# Autodesk Inventor assembly: rat_enclosure
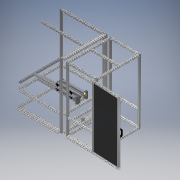
[picture p0: Inventor's stored thumbnail of the model, 180x180]
Saved by Autodesk Inventor 2019 (Build 230136000, 136)
## iProperties
Created: 2018-07-19
Part Number: rat_enclosure
Document SubType Name: Assembly
Designer: Brian
Author: Brian
## Documents named in this file (29)
- C:\Users\bgereke\Desktop\designs\rat_enclosure.iam
- C:\Users\bgereke\Desktop\designs\24in_1010.ipt
- C:\Users\bgereke\Desktop\designs\24in_1020.ipt
- C:\Users\bgereke\Desktop\designs\38in_1010.ipt
- C:\Users\bgereke\Desktop\designs\38in_1020.ipt
- C:\Users\bgereke\Desktop\designs\35in_1010.ipt
- C:\Users\bgereke\Desktop\designs\24in_half_1010.ipt
- C:\Users\bgereke\Desktop\designs\4in_1010.ipt
- C:\Users\bgereke\Desktop\designs\16in_1010.ipt
- C:\Users\bgereke\Desktop\designs\rat_enclosure_top_panel.ipt
- C:\Users\bgereke\Desktop\designs\rat_enclosure_side_panels.ipt
- C:\Users\bgereke\Desktop\designs\rat_enclosure_door_panel.ipt
- C:\Users\bgereke\Desktop\designs\16in_1020.ipt
- C:\Users\bgereke\Desktop\designs\16in_half_1010.ipt
- C:\Users\bgereke\Desktop\designs\arm_enclosure_back_panel.ipt
- C:\Users\bgereke\Desktop\designs\arm_enclosure_top_panel.ipt
- C:\Users\bgereke\Desktop\designs\arm_enclosure_side_panel.ipt
- C:\Users\bgereke\Desktop\designs\arm_enclosure_door_panel.ipt
- C:\Users\bgereke\Desktop\designs\2062\2062.ipt
- C:\Users\bgereke\Desktop\designs\rat_enclosure_slide_panel.ipt
- C:\Users\bgereke\Documents\BSE poster 2019\Gimbal_bot.iam
- C:\Users\bgereke\Desktop\designs\Nord\BRAIN-assembly-complete-model-08-13-18.iam
- C:\Users\bgereke\Desktop\designs\head port\head_port_1.ipt
- C:\Users\bgereke\Desktop\designs\8020_27511\AIS2019\2751-1.iam
- C:\Users\bgereke\Desktop\designs\4in_1020.ipt
- C:\Users\bgereke\Desktop\designs\3310T592_STRUT CHANNEL.ipt
- C:\Users\bgereke\Desktop\designs\confiner_back_panel.ipt
- C:\Users\bgereke\Desktop\designs\confiner_floor.ipt
- C:\Users\bgereke\Desktop\designs\confiner_sliding_panel.ipt
## Components (77 placed, 28 different names)
1. 24in_1010:1 — Flush:3, Mate:5, Mate:6, Flush:12, Flush:14, Mate:18, Flush:45
2. 24in_1010:3 — Flush:3, Mate:5, Mate:6, Flush:13, Flush:25
3. 24in_1020:1 — Flush:25, Flush:34, Mate:30, Flush:104, Flush:166, Mate:114, Mate:150
4. 24in_1010:4 — Mate:17, Mate:20, Flush:36, Flush:37, Mate:31, Flush:42, Flush:130
5. 24in_1010:6 — Flush:22, Flush:28, Mate:26, Mate:27, Flush:29, Flush:131, Mate:134
6. 24in_1020:2 — Mate:25, Flush:30, Flush:35, Flush:57, Mate:82, Mate:102, Mate:132
7. 38in_1010:3 — Flush:12, Flush:13, Flush:14, Flush:22, Mate:20, Flush:27, Mate:24, Mate:27, Flush:129, Mate:88, Mate:156, Flush:196
8. 24in_1010:7 — Mate:17, Mate:18, Flush:20, Flush:27, Mate:24, Flush:43, Mate:87, Mate:182, Flush:234
9. 24in_1010:8 — Flush:20, Flush:33, Mate:29, Flush:73, Flush:272
10. 38in_1020:1 — Flush:28, Mate:25, Mate:26, Flush:29, Flush:30, Flush:33, Flush:34, Mate:29, Flush:35, Mate:30, Flush:74, Flush:100
11. 38in_1020:2 — Flush:36, Flush:37, Mate:31, Flush:40, Flush:41, Mate:33, Mate:34, Flush:46, Mate:35, Flush:54
12. 24in_1010:9 — Flush:40, Flush:41, Flush:42, Mate:33, Flush:55, Flush:56, Flush:177, Mate:133
13. 24in_1010:10 — Flush:43, Mate:34, Flush:54
14. 24in_1020:3 — Flush:45, Flush:46, Mate:35
15. 24in_half_1010:2 — Flush:132, Mate:90, Mate:145
16. 24in_half_1010:1
17. 35in_1010:1 — Mate:91, Mate:144, Flush:183
18. 35in_1010:2
19. 38in_1010:4 — Flush:55, Flush:56, Flush:57, Mate:51, Mate:81, Mate:83, Mate:84, Mate:86
20. 24in_1020:4 — Flush:73, Flush:74, Mate:51, Mate:85, Mate:150, Mate:151, Flush:188, Flush:277, Flush:282, Mate:226
21. 38in_1010:6 — Flush:100, Flush:108, Mate:69, Flush:109, Flush:120, Flush:121, Flush:136, Mate:98, Flush:140, Flush:144
22. 24in_1010:11 — Mate:98, Flush:140, Flush:144, Mate:102, Flush:145, Flush:147, Flush:163
23. 24in_1010:12 — Flush:104, Flush:157, Flush:158, Flush:166, Mate:114
24. 16in_1010:2 — Flush:108, Mate:69, Flush:109
25. 38in_1010:8 — Mate:72, Flush:117, Mate:75, Flush:124, Mate:78, Mate:96, Flush:151, Flush:153, Flush:154, Flush:155, Mate:117, Mate:118, Mate:119
26. 24in_1010:13 — Mate:72, Flush:150, Flush:151, Mate:104, Flush:161, Mate:116, Flush:174, Mate:135
27. 24in_1010:14 — Flush:117, Flush:155, Flush:156, Mate:118, Mate:120, Mate:121
28. 16in_1010:4 — Flush:120, Flush:121, Mate:75, Flush:135, Mate:105, Flush:153, Mate:137
29. 16in_1010:5 — Flush:123, Flush:126, Mate:79, Mate:80, Mate:107, Flush:160, Flush:164
30. 16in_1010:6 — Flush:123, Flush:124, Mate:78
31. 24in_1010:15 — Flush:126, Mate:79, Flush:127, Flush:186
32. 24in_1010:16 — Flush:127, Mate:80, Mate:148, Flush:185
33. rat_enclosure_top_panel:1 — Mate:81, Mate:82, Mate:83
34. rat_enclosure_top_panel:2 — Mate:84, Mate:85, Mate:86, Mate:149, Flush:187
35. rat_enclosure_side_panels:1 — Flush:129, Flush:130, Mate:87, Mate:89
36. rat_enclosure_side_panels:2 — Flush:131, Mate:88, Mate:89
37. rat_enclosure_door_panel:1 — Flush:132, Mate:90, Mate:91
38. arm_enclosure_back_panel:1 — Flush:135, Mate:96, Flush:136, Mate:105, Flush:154
39. 16in_1020:1 — Flush:156, Mate:106, Flush:159, Mate:110, Mate:112, Angle:4
40. 38in_1020:4 — Flush:150, Mate:104, Mate:106, Flush:159, Mate:107, Flush:160, Flush:162, Mate:113, Flush:169
41. 38in_1010:9 — Flush:145, Flush:147, Flush:157, Flush:158, Flush:164, Flush:165, Mate:108
42. 16in_1010:7 — Flush:161, Flush:162, Flush:163, Flush:165, Mate:108, Flush:178, Mate:136
43. 35in_1010:3 — Flush:167, Flush:168, Mate:111, Flush:170
44. 16in_half_1010:1 — Mate:110, Flush:167, Flush:168, Mate:111, Mate:112, Mate:113, Angle:4, Flush:171, Mate:123, Mate:125
45. 16in_half_1010:2 — Flush:169, Flush:170, Flush:171, Flush:172, Mate:115, Flush:173, Mate:143
46. 35in_1010:4 — Flush:172, Mate:115, Flush:173, Mate:124, Mate:142, Flush:182
47. arm_enclosure_top_panel:1 — Mate:116, Flush:174, Mate:117
48. arm_enclosure_side_panel:1 — Mate:119, Mate:120, Mate:121
49. arm_enclosure_door_panel:1 — Mate:123, Mate:124, Mate:125
50. 4in_1010:5
51. 4in_1010:6
52. 24in_1010:17 — Flush:177, Mate:132, Mate:133, Mate:134
53. 16in_1010:8 — Flush:178, Mate:135, Mate:136, Mate:137
54. 2062:1 — Mate:142, Flush:182, Mate:143
55. 2062:2 — Mate:144, Flush:183, Mate:145
56. rat_enclosure_slide_panel:1
57. Gimbal_bot:1 [sub-assembly] — Mate:148, Flush:185, Flush:186
58. BRAIN-assembly-complete-model-08-13-18:1 [sub-assembly] — Mate:149, Flush:187
59. 24in_1010:19 — Mate:151, Flush:188, Flush:252, Flush:272, Mate:242, Mate:243, Flush:298
60. 24in_1010:23 — Mate:156, Flush:196, Mate:227, Flush:283
61. head_port_1:1 — Flush:208, Flush:252, Mate:212, Flush:254, Mate:221, Flush:276, Mate:230, Flush:287
62. head_port_1:2 — Flush:208, Flush:253, Mate:212, Flush:254, Flush:255, Mate:225, Flush:289
63. 24in_1010:24 — Mate:182, Flush:234, Flush:253, Flush:255, Mate:234, Flush:290, Flush:297
64. 2751-1:1 [sub-assembly] — Flush:269, Mate:235, Mate:236, Flush:292
65. 2751-1:2 [sub-assembly] — Flush:269, Mate:237, Flush:293
66. 4in_1010:9 — Mate:221, Flush:276, Flush:277, Flush:281, Mate:228, Mate:239
67. 4in_1010:10 — Mate:233, Mate:234, Flush:290, Flush:292, Flush:293
68. 4in_1020:1 — Flush:281, Flush:282, Mate:225, Mate:226, Flush:284
69. 24in_1010:25 — Mate:227, Flush:283, Flush:284, Mate:235, Mate:236, Mate:237, Flush:291
70. 3310T592_STRUT CHANNEL:1 — Mate:228, Mate:230, Flush:287, Flush:288, Flush:294, Mate:238, Mate:244, Mate:245, Mate:247
71. 3310T592_STRUT CHANNEL:2 — Flush:288, Flush:289, Mate:233, Flush:291, Flush:295, Mate:240, Flush:296
72. confiner_back_panel:1 — Flush:294, Mate:238, Mate:239
73. confiner_back_panel:2 — Flush:295, Mate:240, Flush:296, Flush:299
74. confiner_floor:1 — Flush:297, Mate:242
75. 4in_1020:2 — Mate:243, Mate:244, Flush:298, Mate:246
76. confiner_sliding_panel:1 — Mate:245, Mate:246, Mate:247, Mate:248, Flush:300
77. confiner_sliding_panel:2 — Mate:248, Flush:299, Flush:300
## Relationships (229: Flush 120, Mate 106, Angle 3)
- Flush:3: 24in_1010:1 ↔ 24in_1010:3
- Mate:5: 24in_1010:1 ↔ 24in_1010:3
- Mate:6: 24in_1010:1 ↔ 24in_1010:3
- [Flush]: 24in_1010:4 ↔ 24in_1010:6
- [Mate]: 24in_1010:4 ↔ 24in_1010:6
- [Mate]: 24in_1010:4 ↔ 24in_1010:6
- Flush:12: 24in_1010:1 ↔ 38in_1010:3
- Flush:13: 24in_1010:3 ↔ 38in_1010:3
- Flush:14: 24in_1010:1 ↔ 38in_1010:3
- Mate:17: 24in_1010:4 ↔ 24in_1010:7
- Mate:18: 24in_1010:1 ↔ 24in_1010:7
- Flush:20: 24in_1010:7 ↔ 24in_1010:8
- Flush:22: 24in_1010:6 ↔ 38in_1010:3
- Mate:20: 24in_1010:4 ↔ 38in_1010:3
- Flush:25: 24in_1010:3 ↔ 24in_1020:1
- Flush:27: 38in_1010:3 ↔ 24in_1010:7
- Mate:24: 38in_1010:3 ↔ 24in_1010:7
- Flush:28: 24in_1010:6 ↔ 38in_1020:1
- Mate:25: 24in_1020:2 ↔ 38in_1020:1
- Mate:26: 24in_1010:6 ↔ 38in_1020:1
- Mate:27: 24in_1010:6 ↔ 38in_1010:3
- Flush:29: 24in_1010:6 ↔ 38in_1020:1
- Flush:30: 24in_1020:2 ↔ 38in_1020:1
- Flush:33: 24in_1010:8 ↔ 38in_1020:1
- Flush:34: 24in_1020:1 ↔ 38in_1020:1
- Mate:29: 24in_1010:8 ↔ 38in_1020:1
- Flush:35: 24in_1020:2 ↔ 38in_1020:1
- Mate:30: 24in_1020:1 ↔ 38in_1020:1
- Flush:36: 24in_1010:4 ↔ 38in_1020:2
- Flush:37: 24in_1010:4 ↔ 38in_1020:2
- Mate:31: 24in_1010:4 ↔ 38in_1020:2
- Flush:40: 38in_1020:2 ↔ 24in_1010:9
- Flush:41: 38in_1020:2 ↔ 24in_1010:9
- Flush:42: 24in_1010:4 ↔ 24in_1010:9
- Mate:33: 38in_1020:2 ↔ 24in_1010:9
- Flush:43: 24in_1010:7 ↔ 24in_1010:10
- Mate:34: 38in_1020:2 ↔ 24in_1010:10
- Flush:45: 24in_1010:1 ↔ 24in_1020:3
- Flush:46: 38in_1020:2 ↔ 24in_1020:3
- Mate:35: 38in_1020:2 ↔ 24in_1020:3
- [Flush]: 24in_1010:9 ↔ 24in_half_1010:2
- [Flush]: 24in_half_1010:2 ↔ 24in_half_1010:1
- [Flush]: 24in_half_1010:2 ↔ 24in_half_1010:1
- [Mate]: 24in_1020:3 ↔ 24in_half_1010:1
- [Mate] (1.778 mm): 38in_1020:2 ↔ 24in_half_1010:1
- [Angle] (0 deg): 24in_1020:3 ↔ 24in_half_1010:1
- [Angle] (0 deg): 24in_1020:3 ↔ 24in_half_1010:1
- [Flush]: 24in_half_1010:2 ↔ 35in_1010:1
- [Flush]: 24in_half_1010:2 ↔ 35in_1010:1
- [Mate]: 24in_half_1010:2 ↔ 35in_1010:1
- [Mate]: 24in_half_1010:1 ↔ 35in_1010:2
- [Flush]: 24in_half_1010:2 ↔ 35in_1010:2
- [Flush]: 24in_half_1010:2 ↔ 35in_1010:2
- Flush:54: 38in_1020:2 ↔ 24in_1010:10
- Flush:55: 24in_1010:9 ↔ 38in_1010:4
- Flush:56: 24in_1010:9 ↔ 38in_1010:4
- Flush:57: 24in_1020:2 ↔ 38in_1010:4
- Flush:73: 24in_1010:8 ↔ 24in_1020:4
- Flush:74: 38in_1020:1 ↔ 24in_1020:4
- Mate:51: 38in_1010:4 ↔ 24in_1020:4
- Flush:100: 38in_1020:1 ↔ 38in_1010:6
- Flush:104: 24in_1020:1 ↔ 24in_1010:12
- Flush:108: 38in_1010:6 ↔ 16in_1010:2
- Mate:69: 38in_1010:6 ↔ 16in_1010:2
- Flush:109: 38in_1010:6 ↔ 16in_1010:2
- Mate:72: 38in_1010:8 ↔ 24in_1010:13
- Flush:117: 38in_1010:8 ↔ 24in_1010:14
- Flush:120: 38in_1010:6 ↔ 16in_1010:4
- Flush:121: 38in_1010:6 ↔ 16in_1010:4
- Mate:75: 38in_1010:8 ↔ 16in_1010:4
- Flush:123: 16in_1010:5 ↔ 16in_1010:6
- Flush:124: 38in_1010:8 ↔ 16in_1010:6
- Mate:78: 38in_1010:8 ↔ 16in_1010:6
- Flush:126: 16in_1010:5 ↔ 24in_1010:15
- Mate:79: 16in_1010:5 ↔ 24in_1010:15
- Flush:127: 24in_1010:15 ↔ 24in_1010:16
- Mate:80: 16in_1010:5 ↔ 24in_1010:16
- Mate:81: 38in_1010:4 ↔ rat_enclosure_top_panel:1
- Mate:82: 24in_1020:2 ↔ rat_enclosure_top_panel:1
- Mate:83: 38in_1010:4 ↔ rat_enclosure_top_panel:1
- Mate:84: 38in_1010:4 ↔ rat_enclosure_top_panel:2
- Mate:85: 24in_1020:4 ↔ rat_enclosure_top_panel:2
- Mate:86: 38in_1010:4 ↔ rat_enclosure_top_panel:2
- Flush:129: 38in_1010:3 ↔ rat_enclosure_side_panels:1
- Flush:130: 24in_1010:4 ↔ rat_enclosure_side_panels:1
- Mate:87: 24in_1010:7 ↔ rat_enclosure_side_panels:1
- Flush:131: 24in_1010:6 ↔ rat_enclosure_side_panels:2
- Mate:88: 38in_1010:3 ↔ rat_enclosure_side_panels:2
- Mate:89: rat_enclosure_side_panels:1 ↔ rat_enclosure_side_panels:2
- Flush:132: 24in_half_1010:2 ↔ rat_enclosure_door_panel:1
- Mate:90: 24in_half_1010:2 ↔ rat_enclosure_door_panel:1
- Mate:91: 35in_1010:1 ↔ rat_enclosure_door_panel:1
- Flush:135: 16in_1010:4 ↔ arm_enclosure_back_panel:1
- Mate:96: 38in_1010:8 ↔ arm_enclosure_back_panel:1
- Flush:136: 38in_1010:6 ↔ arm_enclosure_back_panel:1
- Mate:98: 38in_1010:6 ↔ 24in_1010:11
- Flush:140: 38in_1010:6 ↔ 24in_1010:11
- Flush:144: 38in_1010:6 ↔ 24in_1010:11
- Mate:102: 24in_1020:2 ↔ 24in_1010:11
- Flush:145: 24in_1010:11 ↔ 38in_1010:9
- Flush:147: 24in_1010:11 ↔ 38in_1010:9
- Flush:150: 24in_1010:13 ↔ 38in_1020:4
- Flush:151: 38in_1010:8 ↔ 24in_1010:13
- Mate:104: 24in_1010:13 ↔ 38in_1020:4
- Mate:105: 16in_1010:4 ↔ arm_enclosure_back_panel:1
- Flush:153: 38in_1010:8 ↔ 16in_1010:4
- Flush:154: 38in_1010:8 ↔ arm_enclosure_back_panel:1
- Flush:155: 38in_1010:8 ↔ 24in_1010:14
- Flush:156: 24in_1010:14 ↔ 16in_1020:1
- Flush:157: 24in_1010:12 ↔ 38in_1010:9
- Flush:158: 24in_1010:12 ↔ 38in_1010:9
- Mate:106: 16in_1020:1 ↔ 38in_1020:4
- Flush:159: 16in_1020:1 ↔ 38in_1020:4
- Mate:107: 16in_1010:5 ↔ 38in_1020:4
- Flush:160: 16in_1010:5 ↔ 38in_1020:4
- Flush:161: 24in_1010:13 ↔ 16in_1010:7
- Flush:162: 38in_1020:4 ↔ 16in_1010:7
- Flush:163: 24in_1010:11 ↔ 16in_1010:7
- Flush:164: 16in_1010:5 ↔ 38in_1010:9
- Flush:165: 38in_1010:9 ↔ 16in_1010:7
- Mate:108: 38in_1010:9 ↔ 16in_1010:7
- Flush:166: 24in_1020:1 ↔ 24in_1010:12
- Mate:110: 16in_1020:1 ↔ 16in_half_1010:1
- Flush:167: 35in_1010:3 ↔ 16in_half_1010:1
- Flush:168: 35in_1010:3 ↔ 16in_half_1010:1
- Mate:111: 35in_1010:3 ↔ 16in_half_1010:1
- Mate:112: 16in_1020:1 ↔ 16in_half_1010:1
- Mate:113 (2.54 mm): 38in_1020:4 ↔ 16in_half_1010:1
- Angle:4 (0 deg): 16in_1020:1 ↔ 16in_half_1010:1
- Flush:169: 38in_1020:4 ↔ 16in_half_1010:2
- Flush:170: 35in_1010:3 ↔ 16in_half_1010:2
- Flush:171: 16in_half_1010:1 ↔ 16in_half_1010:2
- Mate:114: 24in_1020:1 ↔ 24in_1010:12
- Flush:172: 16in_half_1010:2 ↔ 35in_1010:4
- Mate:115: 16in_half_1010:2 ↔ 35in_1010:4
- Flush:173: 16in_half_1010:2 ↔ 35in_1010:4
- Mate:116: 24in_1010:13 ↔ arm_enclosure_top_panel:1
- Flush:174: 24in_1010:13 ↔ arm_enclosure_top_panel:1
- Mate:117: 38in_1010:8 ↔ arm_enclosure_top_panel:1
- Mate:118: 38in_1010:8 ↔ 24in_1010:14
- Mate:119: 38in_1010:8 ↔ arm_enclosure_side_panel:1
- Mate:120: 24in_1010:14 ↔ arm_enclosure_side_panel:1
- Mate:121: 24in_1010:14 ↔ arm_enclosure_side_panel:1
- Mate:123: 16in_half_1010:1 ↔ arm_enclosure_door_panel:1
- Mate:124: 35in_1010:4 ↔ arm_enclosure_door_panel:1
- Mate:125: 16in_half_1010:1 ↔ arm_enclosure_door_panel:1
- [Flush]: 38in_1010:6 ↔ 4in_1010:5
- [Mate]: 38in_1010:6 ↔ 4in_1010:5
- [Flush]: 24in_1010:12 ↔ 4in_1010:6
- [Mate]: 24in_1010:12 ↔ 4in_1010:6
- [Mate]: 38in_1010:6 ↔ 4in_1010:6
- [Mate]: 38in_1010:9 ↔ 4in_1010:6
- [Mate]: arm_enclosure_top_panel:1 ↔ 4in_1010:5
- [Mate]: 24in_1010:12 ↔ 4in_1010:5
- Flush:177: 24in_1010:9 ↔ 24in_1010:17
- Mate:132: 24in_1020:2 ↔ 24in_1010:17
- Mate:133: 24in_1010:9 ↔ 24in_1010:17
- Mate:134: 24in_1010:6 ↔ 24in_1010:17
- Flush:178: 16in_1010:7 ↔ 16in_1010:8
- Mate:135: 24in_1010:13 ↔ 16in_1010:8
- Mate:136: 16in_1010:7 ↔ 16in_1010:8
- Mate:137: 16in_1010:4 ↔ 16in_1010:8
- Mate:142: 35in_1010:4 ↔ 2062:1
- Flush:182 (-1.27 mm): 35in_1010:4 ↔ 2062:1
- Mate:143 (-482.6 mm): 16in_half_1010:2 ↔ 2062:1
- Mate:144: 35in_1010:1 ↔ 2062:2
- Flush:183 (1.27 mm): 35in_1010:1 ↔ 2062:2
- Mate:145 (-482.6 mm): 24in_half_1010:2 ↔ 2062:2
- Mate:148: 24in_1010:16 ↔ Gimbal_bot:1
- Flush:185: 24in_1010:16 ↔ Gimbal_bot:1
- Flush:186: 24in_1010:15 ↔ Gimbal_bot:1
- Mate:149: rat_enclosure_top_panel:2 ↔ BRAIN-assembly-complete-model-08-13-18:1
- Flush:187: rat_enclosure_top_panel:2 ↔ BRAIN-assembly-complete-model-08-13-18:1
- Mate:150 (204.47 mm): 24in_1020:1 ↔ 24in_1020:4
- Mate:151: 24in_1020:4 ↔ 24in_1010:19
- Flush:188: 24in_1020:4 ↔ 24in_1010:19
- Mate:156: 38in_1010:3 ↔ 24in_1010:23
- Flush:196: 38in_1010:3 ↔ 24in_1010:23
- Flush:208: head_port_1:1 ↔ head_port_1:2
- Mate:182: 24in_1010:7 ↔ 24in_1010:24
- Flush:234: 24in_1010:7 ↔ 24in_1010:24
- Flush:252: 24in_1010:19 ↔ head_port_1:1
- Flush:253: head_port_1:2 ↔ 24in_1010:24
- Mate:212 (38.1 mm): head_port_1:1 ↔ head_port_1:2
- Flush:254: head_port_1:1 ↔ head_port_1:2
- Flush:255 (-88.9 mm): head_port_1:2 ↔ 24in_1010:24
- Flush:269: 2751-1:1 ↔ 2751-1:2
- Flush:272 (-289.7124 mm): 24in_1010:8 ↔ 24in_1010:19
- Mate:221: head_port_1:1 ↔ 4in_1010:9
- Flush:276: head_port_1:1 ↔ 4in_1010:9
- Flush:277: 24in_1020:4 ↔ 4in_1010:9
- Flush:281: 4in_1010:9 ↔ 4in_1020:1
- Flush:282: 24in_1020:4 ↔ 4in_1020:1
- Mate:225: head_port_1:2 ↔ 4in_1020:1
- Mate:226: 24in_1020:4 ↔ 4in_1020:1
- Mate:227: 24in_1010:23 ↔ 24in_1010:25
- Flush:283: 24in_1010:23 ↔ 24in_1010:25
- Flush:284: 4in_1020:1 ↔ 24in_1010:25
- Mate:228: 4in_1010:9 ↔ 3310T592_STRUT CHANNEL:1
- Mate:230 (-1.27 mm): head_port_1:1 ↔ 3310T592_STRUT CHANNEL:1
- Flush:287: head_port_1:1 ↔ 3310T592_STRUT CHANNEL:1
- Flush:288: 3310T592_STRUT CHANNEL:1 ↔ 3310T592_STRUT CHANNEL:2
- Flush:289: head_port_1:2 ↔ 3310T592_STRUT CHANNEL:2
- Mate:233: 4in_1010:10 ↔ 3310T592_STRUT CHANNEL:2
- Mate:234: 24in_1010:24 ↔ 4in_1010:10
- Flush:290: 24in_1010:24 ↔ 4in_1010:10
- Mate:235: 2751-1:1 ↔ 24in_1010:25
- Mate:236: 2751-1:1 ↔ 24in_1010:25
- Mate:237: 2751-1:2 ↔ 24in_1010:25
- Flush:291 (11.2268 mm): 24in_1010:25 ↔ 3310T592_STRUT CHANNEL:2
- Flush:292 (38.354 mm): 2751-1:1 ↔ 4in_1010:10
- Flush:293 (241.681 mm): 2751-1:2 ↔ 4in_1010:10
- Flush:294: 3310T592_STRUT CHANNEL:1 ↔ confiner_back_panel:1
- Mate:238: 3310T592_STRUT CHANNEL:1 ↔ confiner_back_panel:1
- Mate:239: 4in_1010:9 ↔ confiner_back_panel:1
- Flush:295: 3310T592_STRUT CHANNEL:2 ↔ confiner_back_panel:2
- Mate:240: 3310T592_STRUT CHANNEL:2 ↔ confiner_back_panel:2
- Flush:296: 3310T592_STRUT CHANNEL:2 ↔ confiner_back_panel:2
- Flush:297: 24in_1010:24 ↔ confiner_floor:1
- Mate:242: 24in_1010:19 ↔ confiner_floor:1
- Mate:243: 24in_1010:19 ↔ 4in_1020:2
- Mate:244: 3310T592_STRUT CHANNEL:1 ↔ 4in_1020:2
- Flush:298: 24in_1010:19 ↔ 4in_1020:2
- Mate:245: 3310T592_STRUT CHANNEL:1 ↔ confiner_sliding_panel:1
- Mate:246: 4in_1020:2 ↔ confiner_sliding_panel:1
- Mate:247 (2.54 mm): 3310T592_STRUT CHANNEL:1 ↔ confiner_sliding_panel:1
- Mate:248 (57.15 mm): confiner_sliding_panel:1 ↔ confiner_sliding_panel:2
- Flush:299: confiner_back_panel:2 ↔ confiner_sliding_panel:2
- Flush:300: confiner_sliding_panel:1 ↔ confiner_sliding_panel:2
## Named parameters: d12_d6 = 0 mm, d13_d7 = 0 mm, d14_d8 = 0 mm
